# Autodesk Inventor assembly: noga_pre
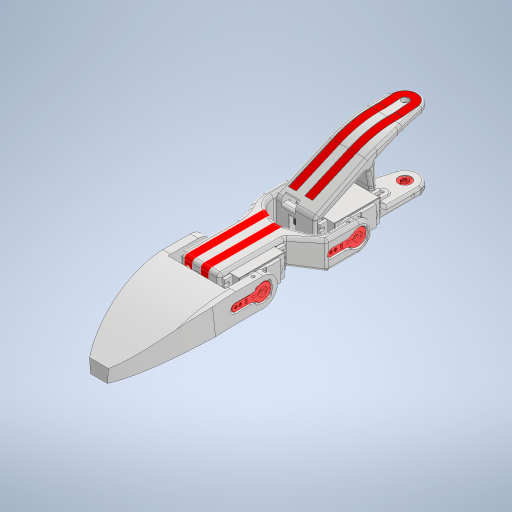
[picture p0: Inventor's stored thumbnail of the model, 512x512]
Saved by Autodesk Inventor 2023.4 (Build 274418000, 418)
## iProperties
Created: 2024-06-27
Part Number: noga_pre
Document SubType Name: Assembly
Designer: kamil
Author: kamil
## Documents named in this file (11)
- E:\PROJECTS_REPOS\Robal-2.0\mechanics\noga_pre.iam
- E:\PROJECTS_REPOS\Robal-2.0\mechanics\Standard-Servo.ipt
- E:\PROJECTS_REPOS\Robal-2.0\mechanics\czlon2_pre.ipt
- E:\PROJECTS_REPOS\Robal-2.0\mechanics\czlon3_pre.ipt
- E:\PROJECTS_REPOS\Robal-2.0\mechanics\czlon4_pre_2.ipt
- E:\PROJECTS_REPOS\Robal-2.0\mechanics\SERVO ARM HORN 25T ALUMINIUM\SERVO ARM HORN 25T ALUMINIUM.ipt
- E:\PROJECTS_REPOS\Robal-2.0\mechanics\czlon_2_wciecie_1.ipt
- E:\PROJECTS_REPOS\Robal-2.0\mechanics\czlon_2_wciecie_2.ipt
- E:\PROJECTS_REPOS\Robal-2.0\mechanics\czlon_2_wciecie_3.ipt
- E:\PROJECTS_REPOS\Robal-2.0\mechanics\czlon_3_wciecie_1.ipt
- E:\PROJECTS_REPOS\Robal-2.0\mechanics\czlon_3_wciecie_2.ipt
## Components (13 placed, 10 different names)
1. Standard-Servo:1 — Zestawiające:9, Zestawiające:11, Mate:24, Mate:25, Mate:26, Angle:4
2. czlon2_pre:1 — Zestawiające:9, Zestawiające:11, Angle:1, Mate:26, Mate:27, Mate:30, Mate:32, Mate:33, Mate:35, Mate:36, Mate:37, Mate:38, Mate:39
3. czlon3_pre:1 — Równoległe:4, Mate:27, Mate:28, Mate:29, Mate:30, Mate:40, Mate:41, Mate:42, Mate:43, Mate:44, Mate:45
4. Standard-Servo:3 — Równoległe:4, Mate:28, Mate:29, Angle:4, Mate:46
5. czlon4_pre_2:1
6. SERVO ARM HORN 25T ALUMINIUM:1 — Angle:1
7. SERVO ARM HORN 25T ALUMINIUM:2 — Mate:24, Mate:25, Flush:5
8. czlon_2_wciecie_1:1 — Mate:32, Mate:33, Mate:37, Angle:3
9. czlon_2_wciecie_2:1 — Mate:35, Mate:36
10. czlon_2_wciecie_3:1 — Mate:38, Mate:39, Angle:3
11. czlon_3_wciecie_1:1 — Mate:40, Mate:41, Mate:42
12. czlon_3_wciecie_2:1 — Mate:43, Mate:44, Mate:45
13. SERVO ARM HORN 25T ALUMINIUM:3 — Flush:5, Mate:46
## Relationships (28: Mate 23, Angle 3, Flush 2)
- Zestawiające:9 [Mate] (1 mm): Standard-Servo:1 ↔ czlon2_pre:1
- Zestawiające:11 [Mate]: Standard-Servo:1 ↔ czlon2_pre:1
- Równoległe:4 [Flush]: czlon3_pre:1 ↔ Standard-Servo:3
- Angle:1 (0 deg): czlon2_pre:1 ↔ SERVO ARM HORN 25T ALUMINIUM:1
- Mate:24: Standard-Servo:1 ↔ SERVO ARM HORN 25T ALUMINIUM:2
- Mate:25: Standard-Servo:1 ↔ SERVO ARM HORN 25T ALUMINIUM:2
- Mate:26: Standard-Servo:1 ↔ czlon2_pre:1
- Mate:27: czlon2_pre:1 ↔ czlon3_pre:1
- Mate:28: czlon3_pre:1 ↔ Standard-Servo:3
- Mate:29: czlon3_pre:1 ↔ Standard-Servo:3
- Mate:30 (2 mm): czlon2_pre:1 ↔ czlon3_pre:1
- Mate:32: czlon2_pre:1 ↔ czlon_2_wciecie_1:1
- Mate:33: czlon2_pre:1 ↔ czlon_2_wciecie_1:1
- Mate:35: czlon2_pre:1 ↔ czlon_2_wciecie_2:1
- Mate:36: czlon2_pre:1 ↔ czlon_2_wciecie_2:1
- Mate:37 (0.1 mm): czlon2_pre:1 ↔ czlon_2_wciecie_1:1
- Mate:38: czlon2_pre:1 ↔ czlon_2_wciecie_3:1
- Mate:39: czlon2_pre:1 ↔ czlon_2_wciecie_3:1
- Angle:3 (180 deg): czlon_2_wciecie_1:1 ↔ czlon_2_wciecie_3:1
- Angle:4 (0 deg): Standard-Servo:1 ↔ Standard-Servo:3
- Mate:40: czlon3_pre:1 ↔ czlon_3_wciecie_1:1
- Mate:41: czlon3_pre:1 ↔ czlon_3_wciecie_1:1
- Mate:42: czlon3_pre:1 ↔ czlon_3_wciecie_1:1
- Mate:43: czlon3_pre:1 ↔ czlon_3_wciecie_2:1
- Mate:44: czlon3_pre:1 ↔ czlon_3_wciecie_2:1
- Mate:45: czlon3_pre:1 ↔ czlon_3_wciecie_2:1
- Flush:5: SERVO ARM HORN 25T ALUMINIUM:2 ↔ SERVO ARM HORN 25T ALUMINIUM:3
- Mate:46: Standard-Servo:3 ↔ SERVO ARM HORN 25T ALUMINIUM:3
